# Autodesk Inventor assembly: HK 2830-1100kv
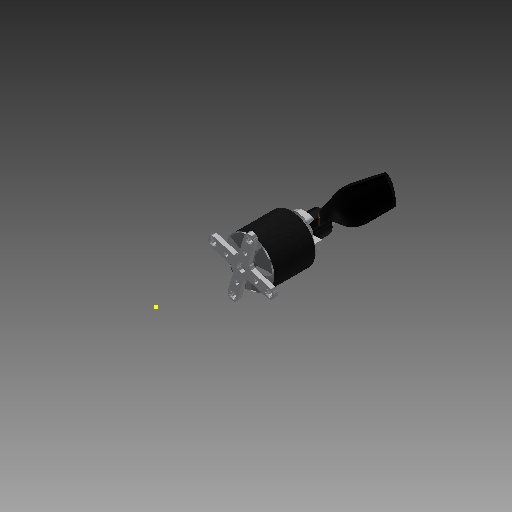
[picture p0: Inventor's stored thumbnail of the model, 512x512]
Saved by Autodesk Inventor 2019 (Build 230136000, 136)
## iProperties
Created: 2014-01-15
Part Number: HK 2830-1100kv
Document SubType Name: Assembly
Designer: Phil
Author: Phil
## Documents named in this file (5)
- C:\Users\varun\Desktop\TSAAssembly\HK 2830-1100kv.iam
- C:\Users\varun\Desktop\TSAAssembly\2830-1100 KV MOTOR.ipt
- C:\Users\varun\Desktop\TSAAssembly\HK 2830 1100 prop adapter.ipt
- C:\Users\varun\Desktop\TSAAssembly\10inchProp.ipt
- C:\Users\varun\Desktop\TSAAssembly\HK 2830 mounting plate.ipt
## Components (4 placed, 4 different names)
1. 2830-1100 KV MOTOR:1 — Mate:1, Mate:2, Mate:3, Flush:1, Mate:6
2. HK 2830 1100 prop adapter:1 — Mate:1, Mate:2, Mate:3, Mate:4, Mate:5
3. 10inchProp:1 — Mate:4, Mate:5
4. HK 2830 mounting plate:1 — Flush:1, Mate:6
## Relationships (7: Mate 6, Flush 1)
- Mate:1: 2830-1100 KV MOTOR:1 ↔ HK 2830 1100 prop adapter:1
- Mate:2: 2830-1100 KV MOTOR:1 ↔ HK 2830 1100 prop adapter:1
- Mate:3: 2830-1100 KV MOTOR:1 ↔ HK 2830 1100 prop adapter:1
- Mate:4: HK 2830 1100 prop adapter:1 ↔ 10inchProp:1
- Mate:5: HK 2830 1100 prop adapter:1 ↔ 10inchProp:1
- Flush:1: 2830-1100 KV MOTOR:1 ↔ HK 2830 mounting plate:1
- Mate:6: 2830-1100 KV MOTOR:1 ↔ HK 2830 mounting plate:1
